# Autodesk Inventor assembly: MCMASTER 1467A109 HINGE
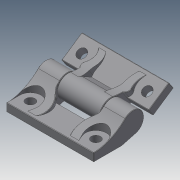
[picture p0: Inventor's stored thumbnail of the model, 180x180]
Saved by Autodesk Inventor 2020.3 (Build 243373000, 373)
## iProperties
RuleStatus: InUse
AfterDocSave0: file://Part Number Cleaner
Created: 2023-03-27
Catalog Web Link: https://www.janelia.org/
Vendor: HHMI: JRC - jET
Document SubType Name: Assembly
Designer: arnoldj
DESIGN DEPARTMENT: HHMI: JRC - jET
ALTERED ITEM PART NUMBER: N/A
ALTERED ITEM VENDOR: N/A
ALTERED ITEM DESCRIPTION: N/A
PART NUMBER - LEGACY: Standard
Author: arnoldj
Revision Number: 0
## Documents named in this file (3)
- C:\_WORKSPACE\DATA\COMMON\McMaster\MCMASTER 1467A109 HINGE.iam
- C:\_WORKSPACE\DATA\COMMON\McMaster\MCMASTER 1467A109_HINGE A..ipt
- C:\_WORKSPACE\DATA\COMMON\McMaster\MCMASTER 1467A109_HINGE B..ipt
## Components (2 placed, 2 different names)
1. MCMASTER 1467A109_HINGE A.:1 — Flush:1, Mate:1
2. MCMASTER 1467A109_HINGE B.:1 — Flush:1, Mate:1
## Relationships (2: Flush 1, Mate 1)
- Flush:1: MCMASTER 1467A109_HINGE A.:1 ↔ MCMASTER 1467A109_HINGE B.:1
- Mate:1: MCMASTER 1467A109_HINGE A.:1 ↔ MCMASTER 1467A109_HINGE B.:1
